# Autodesk Inventor assembly: Assembly
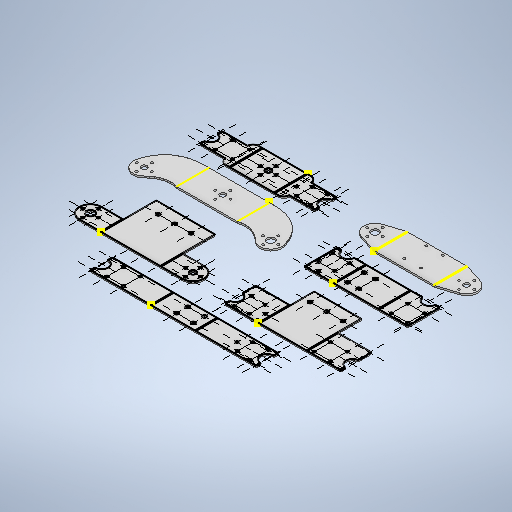
[picture p0: Inventor's stored thumbnail of the model, 512x512]
Saved by Autodesk Inventor 2026.1 (Build 301233000, 233)
## iProperties
Created: 2025-08-15
Part Number: Assembly
Document SubType Name: Assembly
Designer: LG
Author: LG
## Documents named in this file (8)
- C:\Users\LG\Desktop\RHp_Humanoid_ver1\CAM\Arm\Left Arm\1.5T\Assembly\Assembly_left.iam
- C:\Users\LG\Desktop\RHp_Humanoid_ver1\CAM\Arm\Left Arm\1.5T\Part\axis_13_top_frame.ipt
- C:\Users\LG\Desktop\RHp_Humanoid_ver1\CAM\Arm\Left Arm\1.5T\Part\axis_14_bottom_frame.ipt
- C:\Users\LG\Desktop\RHp_Humanoid_ver1\CAM\Arm\Left Arm\1.5T\Part\axis_15_bottom_frame.ipt
- C:\Users\LG\Desktop\RHp_Humanoid_ver1\CAM\Arm\Left Arm\1.5T\Part\axis_16_bottom_frame.ipt
- C:\Users\LG\Desktop\RHp_Humanoid_ver1\CAM\Arm\Left Arm\1.5T\Part\axis_16_top_frame.ipt
- C:\Users\LG\Desktop\RHp_Humanoid_ver1\CAM\Arm\Left Arm\1.5T\Part\axis_17_bottom_frame.ipt
- C:\Users\LG\Desktop\RHp_Humanoid_ver1\CAM\Arm\Left Arm\1.5T\Part\axis_17_top_frame.ipt
## Components (7 placed, 7 different names)
1. axis_13_top_frame:1 — Mate:1, Mate:2, Flush:1, Flush:3, Mate:5, Flush:4, Mate:6, Flush:5, Mate:7, Mate:8, Flush:6, Flush:7, Mate:9, Flush:8, Mate:10, Mate:11, Flush:9, Mate:12, Mate:13, Mate:14, Flush:10
2. axis_14_bottom_frame:1 — Flush:3, Mate:5, Flush:4
3. axis_15_bottom_frame:1 — Mate:13, Mate:14, Flush:10
4. axis_16_bottom_frame:1 — Mate:6, Flush:5, Mate:7
5. axis_16_top_frame:1 — Mate:11, Flush:9, Mate:12
6. axis_17_bottom_frame:1 — Mate:8, Flush:6, Flush:7
7. axis_17_top_frame:1 — Mate:9, Flush:8, Mate:10
## Relationships (21: Mate 12, Flush 9)
- Mate:1: axis_13_top_frame:1
- Mate:2: axis_13_top_frame:1
- Flush:1: axis_13_top_frame:1
- Flush:3: axis_13_top_frame:1 ↔ axis_14_bottom_frame:1
- Mate:5 (45 mm): axis_13_top_frame:1 ↔ axis_14_bottom_frame:1
- Flush:4: axis_13_top_frame:1 ↔ axis_14_bottom_frame:1
- Mate:6 (15 mm): axis_13_top_frame:1 ↔ axis_16_bottom_frame:1
- Flush:5: axis_13_top_frame:1 ↔ axis_16_bottom_frame:1
- Mate:7 (40 mm): axis_13_top_frame:1 ↔ axis_16_bottom_frame:1
- Mate:8 (60 mm): axis_13_top_frame:1 ↔ axis_17_bottom_frame:1
- Flush:6 (-25 mm): axis_13_top_frame:1 ↔ axis_17_bottom_frame:1
- Flush:7: axis_13_top_frame:1 ↔ axis_17_bottom_frame:1
- Mate:9 (60 mm): axis_13_top_frame:1 ↔ axis_17_top_frame:1
- Flush:8: axis_13_top_frame:1 ↔ axis_17_top_frame:1
- Mate:10 (33 mm): axis_13_top_frame:1 ↔ axis_17_top_frame:1
- Mate:11 (125 mm): axis_13_top_frame:1 ↔ axis_16_top_frame:1
- Flush:9: axis_13_top_frame:1 ↔ axis_16_top_frame:1
- Mate:12 (-55 mm): axis_13_top_frame:1 ↔ axis_16_top_frame:1
- Mate:13 (10 mm): axis_13_top_frame:1 ↔ axis_15_bottom_frame:1
- Mate:14 (7 mm): axis_13_top_frame:1 ↔ axis_15_bottom_frame:1
- Flush:10: axis_13_top_frame:1 ↔ axis_15_bottom_frame:1
